# Autodesk Inventor assembly: Ensemble
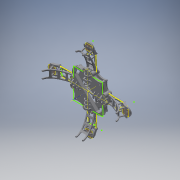
[picture p0: Inventor's stored thumbnail of the model, 180x180]
Saved by Autodesk Inventor 2017 (Build 210142000, 142)
## iProperties
Part Number: Ensemble
Material: Générique
Document SubType Name: Assembly
Designer: Thomas
Author: Thomas
## Documents named in this file (4)
- C:\Users\Thomas\Documents\Modele 3D\Drone\Ensemble.iam
- C:\Users\Thomas\Documents\Modele 3D\Drone\Base.ipt
- C:\Users\Thomas\Documents\Modele 3D\Drone\Ailev3.ipt
- C:\Users\Thomas\Documents\Modele 3D\Drone\Base2.ipt
## Components (7 placed, 3 different names)
1. Base:1 — Placage:16, Placage:18, Affleurement:1, Placage:19, Placage:20, Placage:21
2. Ailev3:1 — Placage:7, Placage:8, Placage:9
3. Ailev3:2 — Placage:5, Placage:12, Placage:13, Placage:18
4. Ailev3:3 — Placage:6, Placage:14, Placage:15
5. Ailev3:4 — Placage:4, Placage:10, Placage:11, Placage:16
6. Base2:1 — Placage:4, Placage:5, Placage:6, Placage:7, Placage:8, Placage:9, Placage:10, Placage:11, Placage:12, Placage:13, Placage:14, Placage:15, Placage:21
7. Base:2 — Affleurement:1, Placage:19, Placage:20
## Relationships (18: Mate 17, Flush 1)
- Placage:4 [Mate]: Ailev3:4 ↔ Base2:1
- Placage:5 [Mate]: Ailev3:2 ↔ Base2:1
- Placage:6 [Mate]: Ailev3:3 ↔ Base2:1
- Placage:7 [Mate]: Ailev3:1 ↔ Base2:1
- Placage:8 [Mate]: Ailev3:1 ↔ Base2:1
- Placage:9 [Mate]: Ailev3:1 ↔ Base2:1
- Placage:10 [Mate]: Ailev3:4 ↔ Base2:1
- Placage:11 [Mate]: Ailev3:4 ↔ Base2:1
- Placage:12 [Mate]: Ailev3:2 ↔ Base2:1
- Placage:13 [Mate]: Ailev3:2 ↔ Base2:1
- Placage:14 [Mate]: Ailev3:3 ↔ Base2:1
- Placage:15 [Mate]: Ailev3:3 ↔ Base2:1
- Placage:16 [Mate]: Base:1 ↔ Ailev3:4
- Placage:18 [Mate]: Base:1 ↔ Ailev3:2
- Affleurement:1 [Flush]: Base:1 ↔ Base:2
- Placage:19 [Mate]: Base:1 ↔ Base:2
- Placage:20 [Mate]: Base:1 ↔ Base:2
- Placage:21 [Mate]: Base:1 ↔ Base2:1
